# Autodesk Inventor assembly: Glue Reservoir Plate - V2
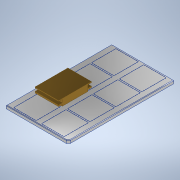
[picture p0: Inventor's stored thumbnail of the model, 180x180]
Saved by Autodesk Inventor 2022 (Build 260153000, 153)
## iProperties
Created: 2022-02-14
Part Number: Glue Reservoir Plate - V2
Document SubType Name: Assembly
Designer: Caleb
Author: Caleb
## Documents named in this file (3)
- C:\Users\Caleb\Desktop\nebraska-silicon-lab\Hardware\ETL\Module Assembly\Glue Reservoir Plate - V2\Glue Reservoir Plate - V2.iam
- C:\Users\Caleb\Desktop\nebraska-silicon-lab\Hardware\ETL\Module Assembly\Glue Stamp - V2\Stamp Assembly - V2.iam
- C:\Users\Caleb\Desktop\nebraska-silicon-lab\Hardware\ETL\Module Assembly\Glue Reservoir Plate - V2\Glue Reservoir Plate - V2.ipt
## Components (2 placed, 2 different names)
1. Stamp Assembly - V2:1 [sub-assembly] — Mate:1
2. Glue Reservoir Plate - V2:1 — Mate:1
## Relationships (1: Mate 1)
- Mate:1: Stamp Assembly - V2:1 ↔ Glue Reservoir Plate - V2:1
